# Autodesk Inventor assembly: X-Anchor
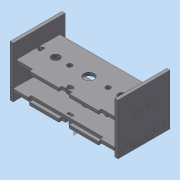
[picture p0: Inventor's stored thumbnail of the model, 180x180]
Saved by Autodesk Inventor 2016 SP1 (Build 200210100, 210)
## iProperties
Created: 2016-02-24
Part Number: X-Anchor
Document SubType Name: Assembly
Designer: Mohamed A.
Author: Mohamed A.
## Documents named in this file (5)
- C:\Users\Mohamed\Documents\inventor\StemCellsPlatform\Laser Cut\X-Anchor\Mirrored\X-Anchor.iam
- C:\Users\Mohamed\Documents\inventor\StemCellsPlatform\Laser Cut\X-Anchor\Mirrored\X-Anchor_Front-Outer.ipt
- C:\Users\Mohamed\Documents\inventor\StemCellsPlatform\Flanges\UFL08 -Housing.ipt
- C:\Users\Mohamed\Documents\inventor\StemCellsPlatform\Laser Cut\X-Anchor\Mirrored\X-Anchor_Front-Inner.ipt
- C:\Users\Mohamed\Documents\inventor\StemCellsPlatform\Laser Cut\X-Anchor\Mirrored\X-Anchor_Front-Side.ipt
## Components (6 placed, 4 different names)
1. UFL08 -Housing:1 — Mate:4
2. X-Anchor_Front-Outer:2 — Flush:5, Flush:6
3. X-Anchor_Front-Side:1 — Flush:6, Flush:8, Flush:9, Flush:10
4. X-Anchor_Front-Side:2 — Flush:1, Flush:2, Flush:7, Flush:8, Flush:9
5. X-Anchor_Front-Inner:3 — Flush:1, Flush:2, Flush:3, Mate:1, Flush:4
6. X-Anchor_Front-Outer:3 — Flush:3, Mate:1, Flush:4, Flush:5, Mate:4, Flush:7, Flush:10
## Relationships (12: Flush 10, Mate 2)
- Flush:1: X-Anchor_Front-Side:2 ↔ X-Anchor_Front-Inner:3
- Flush:2: X-Anchor_Front-Side:2 ↔ X-Anchor_Front-Inner:3
- Flush:3: X-Anchor_Front-Inner:3 ↔ X-Anchor_Front-Outer:3
- Mate:1: X-Anchor_Front-Inner:3 ↔ X-Anchor_Front-Outer:3
- Flush:4: X-Anchor_Front-Inner:3 ↔ X-Anchor_Front-Outer:3
- Flush:5: X-Anchor_Front-Outer:2 ↔ X-Anchor_Front-Outer:3
- Flush:6: X-Anchor_Front-Outer:2 ↔ X-Anchor_Front-Side:1
- Mate:4: UFL08 -Housing:1 ↔ X-Anchor_Front-Outer:3
- Flush:7 (5 mm): X-Anchor_Front-Side:2 ↔ X-Anchor_Front-Outer:3
- Flush:8: X-Anchor_Front-Side:1 ↔ X-Anchor_Front-Side:2
- Flush:9: X-Anchor_Front-Side:1 ↔ X-Anchor_Front-Side:2
- Flush:10: X-Anchor_Front-Side:1 ↔ X-Anchor_Front-Outer:3
